# Autodesk Inventor assembly: Hond
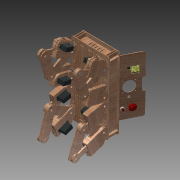
[picture p0: Inventor's stored thumbnail of the model, 180x180]
Saved by Autodesk Inventor 2015 (Build 190159000, 159)
## iProperties
Created: 2015-12-19
Part Number: Hond
Document SubType Name: Assembly
Designer: david
Author: david
## Documents named in this file (10)
- Z:\gip\Inventor\generatie 7\Hond.iam
- Z:\gip\Inventor\generatie 7\Frame\Frame.iam
- Z:\gip\Inventor\generatie 7\Beenen\onderbeen\Onderbeen.iam
- Z:\gip\Inventor\generatie 7\Motor\Motor.iam
- Z:\gip\Inventor\generatie 7\Beenen\MidRing\MidRing.ipt
- Z:\gip\Inventor\generatie 7\Beenen\onderbeen\onderpoot.iam
- Z:\gip\Inventor\generatie 7\motor v2\motor.iam
- Z:\gip\Inventor\generatie 7\Motor\motor_MIROR.iam
- Z:\gip\Inventor\generatie 7\motor v2\motor_MIROR1.iam
- Z:\gip\Inventor\generatie 7\Vijs.ipt
## Components (21 placed, 9 different names)
1. Frame:1 [sub-assembly] — Mate:3, Mate:4, Mate:5, Mate:6, Mate:7, Mate:8, Mate:9, Mate:13, Mate:14, Mate:15, Mate:16, Mate:19, Mate:25, Mate:26, Mate:28, Mate:29, Mate:45, Mate:47, Mate:48, Mate:49, Mate:50, Mate:52, Mate:53, Mate:56, Mate:57, Mate:66, Mate:67, Mate:69, Mate:70
2. Onderbeen:1 [sub-assembly] — Mate:3, Mate:9, Mate:27
3. Onderbeen:2 [sub-assembly] — Mate:4, Mate:41, Mate:42, Mate:48
4. Onderbeen:3 [sub-assembly] — Mate:6, Mate:7, Mate:30, Mate:40
5. Onderbeen:4 [sub-assembly] — Mate:5, Mate:8, Mate:38, Mate:59
6. MidRing:3 — Mate:14, Mate:15
7. MidRing:4 — Mate:13, Mate:16
8. Motor:1 [sub-assembly] — Mate:25, Mate:26, Mate:27, Mate:43, Mate:44
9. Motor:2 [sub-assembly] — Mate:28, Mate:29, Mate:30, Mate:39
10. onderpoot:1 [sub-assembly] — Mate:38, Mate:46, Mate:58
11. onderpoot:2 [sub-assembly] — Mate:39, Mate:40, Mate:65
12. onderpoot:3 [sub-assembly] — Mate:41, Mate:42, Mate:54, Mate:55
13. onderpoot:4 [sub-assembly] — Mate:43, Mate:44, Mate:68, Mate:73, Mate:74
14. motor:1 [sub-assembly] — Mate:45, Mate:46, Mate:47
15. motor:2 [sub-assembly] — Mate:49, Mate:50, Mate:55
16. motor_MIROR:1 [sub-assembly] — Mate:52, Mate:53, Mate:54
17. motor_MIROR:2 [sub-assembly] — Mate:56, Mate:57, Mate:58, Mate:59
18. motor_MIROR1:1 [sub-assembly] — Mate:65, Mate:66, Mate:67
19. motor_MIROR1:2 [sub-assembly] — Mate:68, Mate:69, Mate:70, Mate:71, Mate:72
20. Vijs:1 — Mate:71, Mate:72
21. Vijs:2 — Mate:73, Mate:74
## Relationships (49: Mate 49)
- Mate:3: Frame:1 ↔ Onderbeen:1
- Mate:4: Frame:1 ↔ Onderbeen:2
- Mate:5: Frame:1 ↔ Onderbeen:4
- Mate:6: Frame:1 ↔ Onderbeen:3
- Mate:7: Frame:1 ↔ Onderbeen:3
- Mate:8: Frame:1 ↔ Onderbeen:4
- Mate:9: Frame:1 ↔ Onderbeen:1
- Mate:13: Frame:1 ↔ MidRing:4
- Mate:14: Frame:1 ↔ MidRing:3
- Mate:15: Frame:1 ↔ MidRing:3
- Mate:16: Frame:1 ↔ MidRing:4
- Mate:19: Frame:1
- Mate:25: Frame:1 ↔ Motor:1
- Mate:26: Frame:1 ↔ Motor:1
- Mate:27: Onderbeen:1 ↔ Motor:1
- Mate:28: Frame:1 ↔ Motor:2
- Mate:29: Frame:1 ↔ Motor:2
- Mate:30: Onderbeen:3 ↔ Motor:2
- Mate:38: Onderbeen:4 ↔ onderpoot:1
- Mate:39: Motor:2 ↔ onderpoot:2
- Mate:40: Onderbeen:3 ↔ onderpoot:2
- Mate:41: Onderbeen:2 ↔ onderpoot:3
- Mate:42: Onderbeen:2 ↔ onderpoot:3
- Mate:43: Motor:1 ↔ onderpoot:4
- Mate:44: Motor:1 ↔ onderpoot:4
- Mate:45: Frame:1 ↔ motor:1
- Mate:46: onderpoot:1 ↔ motor:1
- Mate:47: Frame:1 ↔ motor:1
- Mate:48: Frame:1 ↔ Onderbeen:2
- Mate:49: Frame:1 ↔ motor:2
- Mate:50: Frame:1 ↔ motor:2
- Mate:52: Frame:1 ↔ motor_MIROR:1
- Mate:53: Frame:1 ↔ motor_MIROR:1
- Mate:54: onderpoot:3 ↔ motor_MIROR:1
- Mate:55: onderpoot:3 ↔ motor:2
- Mate:56: Frame:1 ↔ motor_MIROR:2
- Mate:57: Frame:1 ↔ motor_MIROR:2
- Mate:58: onderpoot:1 ↔ motor_MIROR:2
- Mate:59: Onderbeen:4 ↔ motor_MIROR:2
- Mate:65: onderpoot:2 ↔ motor_MIROR1:1
- Mate:66: Frame:1 ↔ motor_MIROR1:1
- Mate:67: Frame:1 ↔ motor_MIROR1:1
- Mate:68: onderpoot:4 ↔ motor_MIROR1:2
- Mate:69: Frame:1 ↔ motor_MIROR1:2
- Mate:70: Frame:1 ↔ motor_MIROR1:2
- Mate:71: motor_MIROR1:2 ↔ Vijs:1
- Mate:72: motor_MIROR1:2 ↔ Vijs:1
- Mate:73: onderpoot:4 ↔ Vijs:2
- Mate:74: onderpoot:4 ↔ Vijs:2
